# Autodesk Inventor assembly: Chuck Assembly
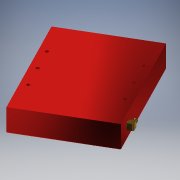
[picture p0: Inventor's stored thumbnail of the model, 180x180]
Saved by Autodesk Inventor 2019.4 (Build 234330000, 330)
## iProperties
Created: 2021-01-11
Part Number: Chuck Assembly
Document SubType Name: Assembly
Designer: caleb
Author: caleb
## Documents named in this file (5)
- C:\Users\cfang\Desktop\nebraska-silicon-lab\CAD\ETL\Module Assembly\Chuck\Chuck Assembly.iam
- C:\Users\cfang\Desktop\nebraska-silicon-lab\CAD\ETL\Module Assembly\Chuck\Chuck.ipt
- C:\Users\cfang\Desktop\nebraska-silicon-lab\CAD\ETL\Module Assembly\Chuck\90128A212_ZNC-PLTD ALLOY STL SCKT HEAD CAP SCREW.ipt
- C:\Users\cfang\Desktop\nebraska-silicon-lab\CAD\ETL\Module Assembly\Chuck\44555K151_BRASS BARBED TUBE FITTING FOR VACUUM.ipt
- C:\Users\cfang\Desktop\nebraska-silicon-lab\CAD\ETL\Module Assembly\Chuck\4464K562_TYPE 304 STAINLESS STL THREADED PIPE FITTING.ipt
## Components (6 placed, 4 different names)
1. Chuck:1 — Insert:1, Insert:2, Insert:3, Insert:6, Insert:7
2. 90128A212_ZNC-PLTD ALLOY STL SCKT HEAD CAP SCREW:1 — Insert:2
3. 90128A212_ZNC-PLTD ALLOY STL SCKT HEAD CAP SCREW:2 — Insert:3
4. 90128A212_ZNC-PLTD ALLOY STL SCKT HEAD CAP SCREW:3 — Insert:1
5. 44555K151_BRASS BARBED TUBE FITTING FOR VACUUM:1 — Insert:7
6. 4464K562_TYPE 304 STAINLESS STL THREADED PIPE FITTING:1 — Insert:6
## Relationships (5: Insert 5)
- Insert:1: Chuck:1 ↔ 90128A212_ZNC-PLTD ALLOY STL SCKT HEAD CAP SCREW:3
- Insert:2: Chuck:1 ↔ 90128A212_ZNC-PLTD ALLOY STL SCKT HEAD CAP SCREW:1
- Insert:3: Chuck:1 ↔ 90128A212_ZNC-PLTD ALLOY STL SCKT HEAD CAP SCREW:2
- Insert:6 (-10.668 mm): Chuck:1 ↔ 4464K562_TYPE 304 STAINLESS STL THREADED PIPE FITTING:1
- Insert:7: Chuck:1 ↔ 44555K151_BRASS BARBED TUBE FITTING FOR VACUUM:1
